# Autodesk Inventor assembly: BoardShiftRegisters
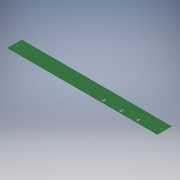
[picture p0: Inventor's stored thumbnail of the model, 180x180]
Saved by Autodesk Inventor 2019.3 (Build 233278000, 278)
## iProperties
Company: Open CASCADE
Created: 2019-02-10
Part Number: BoardShiftRegisters
Material: Generisch
Description: Open CASCADE Model
Document SubType Name: Assembly
Designer: Jonas
Authority: Unknown
Sending System: Open CASCADE 6.8
Preprocessor: Open CASCADE STEP processor 6.8
Title: Open CASCADE Shape Model
Author: Author
## Documents named in this file (85)
- C:\Users\Jonas\Desktop\RGBCube-v2\CAD\PCBs\BoardShiftRegisters.iam
- C:\Users\Jonas\Desktop\RGBCube-v2\CAD\PCBs\BoardBoard.iam
- C:\Users\Jonas\Desktop\RGBCube-v2\CAD\PCBs\BoardT24.iam
- C:\Users\Jonas\Desktop\RGBCube-v2\CAD\PCBs\BoardT23.iam
- C:\Users\Jonas\Desktop\RGBCube-v2\CAD\PCBs\BoardT22.iam
- C:\Users\Jonas\Desktop\RGBCube-v2\CAD\PCBs\BoardT21.iam
- C:\Users\Jonas\Desktop\RGBCube-v2\CAD\PCBs\BoardT20.iam
- C:\Users\Jonas\Desktop\RGBCube-v2\CAD\PCBs\BoardT19.iam
- C:\Users\Jonas\Desktop\RGBCube-v2\CAD\PCBs\BoardT18.iam
- C:\Users\Jonas\Desktop\RGBCube-v2\CAD\PCBs\BoardT17.iam
- C:\Users\Jonas\Desktop\RGBCube-v2\CAD\PCBs\BoardT16.iam
- C:\Users\Jonas\Desktop\RGBCube-v2\CAD\PCBs\BoardT15.iam
- C:\Users\Jonas\Desktop\RGBCube-v2\CAD\PCBs\BoardT14.iam
- C:\Users\Jonas\Desktop\RGBCube-v2\CAD\PCBs\BoardT13.iam
- C:\Users\Jonas\Desktop\RGBCube-v2\CAD\PCBs\BoardT12.iam
- C:\Users\Jonas\Desktop\RGBCube-v2\CAD\PCBs\BoardT11.iam
- C:\Users\Jonas\Desktop\RGBCube-v2\CAD\PCBs\BoardT10.iam
- C:\Users\Jonas\Desktop\RGBCube-v2\CAD\PCBs\BoardT9.iam
- C:\Users\Jonas\Desktop\RGBCube-v2\CAD\PCBs\BoardR48.iam
- C:\Users\Jonas\Desktop\RGBCube-v2\CAD\PCBs\BoardR47.iam
- C:\Users\Jonas\Desktop\RGBCube-v2\CAD\PCBs\BoardR46.iam
- C:\Users\Jonas\Desktop\RGBCube-v2\CAD\PCBs\BoardR45.iam
- C:\Users\Jonas\Desktop\RGBCube-v2\CAD\PCBs\BoardR44.iam
- C:\Users\Jonas\Desktop\RGBCube-v2\CAD\PCBs\BoardR43.iam
- C:\Users\Jonas\Desktop\RGBCube-v2\CAD\PCBs\BoardR42.iam
- C:\Users\Jonas\Desktop\RGBCube-v2\CAD\PCBs\BoardR41.iam
- C:\Users\Jonas\Desktop\RGBCube-v2\CAD\PCBs\BoardR40.iam
- C:\Users\Jonas\Desktop\RGBCube-v2\CAD\PCBs\BoardR39.iam
- C:\Users\Jonas\Desktop\RGBCube-v2\CAD\PCBs\BoardR38.iam
- C:\Users\Jonas\Desktop\RGBCube-v2\CAD\PCBs\BoardR37.iam
- C:\Users\Jonas\Desktop\RGBCube-v2\CAD\PCBs\BoardR36.iam
- C:\Users\Jonas\Desktop\RGBCube-v2\CAD\PCBs\BoardR35.iam
- C:\Users\Jonas\Desktop\RGBCube-v2\CAD\PCBs\BoardR34.iam
- C:\Users\Jonas\Desktop\RGBCube-v2\CAD\PCBs\BoardR33.iam
- C:\Users\Jonas\Desktop\RGBCube-v2\CAD\PCBs\BoardR32.iam
- C:\Users\Jonas\Desktop\RGBCube-v2\CAD\PCBs\BoardR31.iam
- C:\Users\Jonas\Desktop\RGBCube-v2\CAD\PCBs\BoardR30.iam
- C:\Users\Jonas\Desktop\RGBCube-v2\CAD\PCBs\BoardR29.iam
- C:\Users\Jonas\Desktop\RGBCube-v2\CAD\PCBs\BoardR28.iam
- C:\Users\Jonas\Desktop\RGBCube-v2\CAD\PCBs\BoardR27.iam
- C:\Users\Jonas\Desktop\RGBCube-v2\CAD\PCBs\BoardR26.iam
- C:\Users\Jonas\Desktop\RGBCube-v2\CAD\PCBs\BoardR25.iam
- C:\Users\Jonas\Desktop\RGBCube-v2\CAD\PCBs\BoardR24.iam
- C:\Users\Jonas\Desktop\RGBCube-v2\CAD\PCBs\BoardR23.iam
- C:\Users\Jonas\Desktop\RGBCube-v2\CAD\PCBs\BoardR22.iam
- C:\Users\Jonas\Desktop\RGBCube-v2\CAD\PCBs\BoardR21.iam
- C:\Users\Jonas\Desktop\RGBCube-v2\CAD\PCBs\BoardR20.iam
- C:\Users\Jonas\Desktop\RGBCube-v2\CAD\PCBs\BoardR19.iam
- C:\Users\Jonas\Desktop\RGBCube-v2\CAD\PCBs\BoardR18.iam
- C:\Users\Jonas\Desktop\RGBCube-v2\CAD\PCBs\BoardR17.iam
- C:\Users\Jonas\Desktop\RGBCube-v2\CAD\PCBs\BoardT8.iam
- C:\Users\Jonas\Desktop\RGBCube-v2\CAD\PCBs\BoardT7.iam
- C:\Users\Jonas\Desktop\RGBCube-v2\CAD\PCBs\BoardT6.iam
- C:\Users\Jonas\Desktop\RGBCube-v2\CAD\PCBs\BoardT5.iam
- C:\Users\Jonas\Desktop\RGBCube-v2\CAD\PCBs\BoardT4.iam
- C:\Users\Jonas\Desktop\RGBCube-v2\CAD\PCBs\BoardT3.iam
- C:\Users\Jonas\Desktop\RGBCube-v2\CAD\PCBs\BoardT2.iam
- C:\Users\Jonas\Desktop\RGBCube-v2\CAD\PCBs\BoardT1.iam
- C:\Users\Jonas\Desktop\RGBCube-v2\CAD\PCBs\BoardR16.iam
- C:\Users\Jonas\Desktop\RGBCube-v2\CAD\PCBs\BoardR15.iam
- C:\Users\Jonas\Desktop\RGBCube-v2\CAD\PCBs\BoardR14.iam
- C:\Users\Jonas\Desktop\RGBCube-v2\CAD\PCBs\BoardR13.iam
- C:\Users\Jonas\Desktop\RGBCube-v2\CAD\PCBs\BoardR12.iam
- C:\Users\Jonas\Desktop\RGBCube-v2\CAD\PCBs\BoardR11.iam
- C:\Users\Jonas\Desktop\RGBCube-v2\CAD\PCBs\BoardR10.iam
- C:\Users\Jonas\Desktop\RGBCube-v2\CAD\PCBs\BoardR9.iam
- C:\Users\Jonas\Desktop\RGBCube-v2\CAD\PCBs\BoardR8.iam
- C:\Users\Jonas\Desktop\RGBCube-v2\CAD\PCBs\BoardR7.iam
- C:\Users\Jonas\Desktop\RGBCube-v2\CAD\PCBs\BoardR6.iam
- C:\Users\Jonas\Desktop\RGBCube-v2\CAD\PCBs\BoardR5.iam
- C:\Users\Jonas\Desktop\RGBCube-v2\CAD\PCBs\BoardR4.iam
- C:\Users\Jonas\Desktop\RGBCube-v2\CAD\PCBs\BoardR3.iam
- C:\Users\Jonas\Desktop\RGBCube-v2\CAD\PCBs\BoardR2.iam
- C:\Users\Jonas\Desktop\RGBCube-v2\CAD\PCBs\BoardR1.iam
- C:\Users\Jonas\Desktop\RGBCube-v2\CAD\PCBs\BoardSR3.iam
- C:\Users\Jonas\Desktop\RGBCube-v2\CAD\PCBs\BoardSR2.iam
- C:\Users\Jonas\Desktop\RGBCube-v2\CAD\PCBs\BoardSR1.iam
- C:\Users\Jonas\Desktop\RGBCube-v2\CAD\PCBs\BoardP1.iam
- C:\Users\Jonas\Desktop\RGBCube-v2\CAD\PCBs\BoardC6.iam
- C:\Users\Jonas\Desktop\RGBCube-v2\CAD\PCBs\BoardC5.iam
- C:\Users\Jonas\Desktop\RGBCube-v2\CAD\PCBs\BoardC4.iam
- C:\Users\Jonas\Desktop\RGBCube-v2\CAD\PCBs\BoardC3.iam
- C:\Users\Jonas\Desktop\RGBCube-v2\CAD\PCBs\BoardC2.iam
- C:\Users\Jonas\Desktop\RGBCube-v2\CAD\PCBs\BoardC1.iam
- C:\Users\Jonas\Desktop\RGBCube-v2\CAD\PCBs\BoardShiftRegisters\AIP\Kabel und Kabelbaum\BoardShiftRegisters.Kabelbaum1.iam
## Components (84 placed, 84 different names)
1. Board_280 [sub-assembly]
2. T24_282 [sub-assembly]
3. T23_284 [sub-assembly]
4. T22_286 [sub-assembly]
5. T21_288 [sub-assembly]
6. T20_290 [sub-assembly]
7. T19_292 [sub-assembly]
8. T18_294 [sub-assembly]
9. T17_296 [sub-assembly]
10. T16_298 [sub-assembly]
11. T15_300 [sub-assembly]
12. T14_302 [sub-assembly]
13. T13_304 [sub-assembly]
14. T12_306 [sub-assembly]
15. T11_308 [sub-assembly]
16. T10_310 [sub-assembly]
17. T9_312 [sub-assembly]
18. R48_318 [sub-assembly]
19. R47_322 [sub-assembly]
20. R46_326 [sub-assembly]
21. R45_330 [sub-assembly]
22. R44_334 [sub-assembly]
23. R43_338 [sub-assembly]
24. R42_342 [sub-assembly]
25. R41_346 [sub-assembly]
26. R40_350 [sub-assembly]
27. R39_354 [sub-assembly]
28. R38_358 [sub-assembly]
29. R37_362 [sub-assembly]
30. R36_366 [sub-assembly]
31. R35_370 [sub-assembly]
32. R34_374 [sub-assembly]
33. R33_378 [sub-assembly]
34. R32_382 [sub-assembly]
35. R31_386 [sub-assembly]
36. R30_390 [sub-assembly]
37. R29_394 [sub-assembly]
38. R28_398 [sub-assembly]
39. R27_402 [sub-assembly]
40. R26_406 [sub-assembly]
41. R25_410 [sub-assembly]
42. R24_414 [sub-assembly]
43. R23_418 [sub-assembly]
44. R22_422 [sub-assembly]
45. R21_426 [sub-assembly]
46. R20_430 [sub-assembly]
47. R19_434 [sub-assembly]
48. R18_438 [sub-assembly]
49. R17_442 [sub-assembly]
50. T8_444 [sub-assembly]
51. T7_446 [sub-assembly]
52. T6_448 [sub-assembly]
53. T5_450 [sub-assembly]
54. T4_452 [sub-assembly]
55. T3_454 [sub-assembly]
56. T2_456 [sub-assembly]
57. T1_458 [sub-assembly]
58. R16_462 [sub-assembly]
59. R15_466 [sub-assembly]
60. R14_470 [sub-assembly]
61. R13_474 [sub-assembly]
62. R12_478 [sub-assembly]
63. R11_482 [sub-assembly]
64. R10_486 [sub-assembly]
65. R9_490 [sub-assembly]
66. R8_494 [sub-assembly]
67. R7_498 [sub-assembly]
68. R6_502 [sub-assembly]
69. R5_506 [sub-assembly]
70. R4_510 [sub-assembly]
71. R3_514 [sub-assembly]
72. R2_518 [sub-assembly]
73. R1_522 [sub-assembly]
74. SR3_524 [sub-assembly]
75. SR2_526 [sub-assembly]
76. SR1_528 [sub-assembly]
77. P1_530 [sub-assembly] — Passend:1
78. C6_536 [sub-assembly]
79. C5_540 [sub-assembly]
80. C4_544 [sub-assembly]
81. C3_548 [sub-assembly]
82. C2_552 [sub-assembly]
83. C1_556 [sub-assembly]
84. Kabelbaum1 [sub-assembly]
## Relationships (1: Mate 1)
- Passend:1 [Mate]: P1_530
